# Autodesk Inventor assembly: 旋转器 小
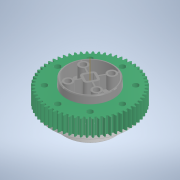
[picture p0: Inventor's stored thumbnail of the model, 180x180]
Saved by Autodesk Inventor 2020 (Build 240168000, 168)
## iProperties
Created: 2019-06-10
Part Number: 旋转器 小
Document SubType Name: Assembly
Designer: aresp
Author: aresp
## Documents named in this file (3)
- C:\Users\aresp\Documents\Vault\常用部件库\vex原厂部件\旋转器 小.iam
- C:\Users\aresp\Documents\Inventor\Content Center Files\R2020\zh-CN\旋转器 小 内层\常规.ipt
- C:\Users\aresp\Documents\Inventor\Content Center Files\R2020\zh-CN\旋转器 小 外层\常规.ipt
## Components (2 placed, 2 different names)
1. 旋转器 小 内层 常规:1 — 配合:1, 配合:2
2. 旋转器 小 外层 常规:1 — 配合:1, 配合:2
## Relationships (2: Mate 2)
- 配合:1 [Mate] (1.0287 mm): 旋转器 小 内层 常规:1 ↔ 旋转器 小 外层 常规:1
- 配合:2 [Mate]: 旋转器 小 内层 常规:1 ↔ 旋转器 小 外层 常规:1
